# Autodesk Inventor assembly: Robot Self Driving 1
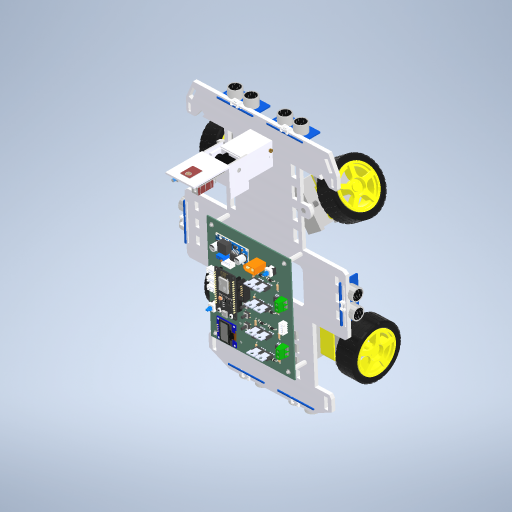
[picture p0: Inventor's stored thumbnail of the model, 512x512]
Saved by Autodesk Inventor 2023 (Build 270158000, 158)
## iProperties
Created: 2025-05-21
Part Number: Robot Self Driving 1
Document SubType Name: Assembly
Designer: ASUS
Author: ASUS
## Documents named in this file (14)
- D:\Backup C\Documents\Inventor\PMLDCAPSTONE\Robot Self Driving 1.iam
- D:\Backup C\Documents\Inventor\PMLDCAPSTONE\Robot_PMLD 1.ipt
- D:\Backup C\Documents\Inventor\PMLDCAPSTONE\Casis Kiri Roda.ipt
- D:\Backup C\Documents\Inventor\PMLDCAPSTONE\Mounting Belakang.ipt
- D:\Backup C\Documents\Inventor\PMLDCAPSTONE\RODA\Roda.iam
- D:\Backup C\Documents\Inventor\PMLDCAPSTONE\Chasis Depan Roda Kiri.ipt
- D:\Backup C\Documents\Inventor\PMLDCAPSTONE\Mounting Depan.ipt
- D:\Backup C\Documents\Inventor\PMLDCAPSTONE\Gearbox\3-6V DC Gearbox Electromotor_MIR.iam
- D:\Backup C\Documents\Inventor\PMLDCAPSTONE\standoff-male-male-m3-1.snapshot.2\3d models\Standoff M3 M-M H 20mm.ipt
- D:\Backup C\Documents\Inventor\PMLDCAPSTONE\Mur Kamera.ipt
- D:\Backup C\Documents\Inventor\PMLDCAPSTONE\Komponen PCB 1.ipt
- D:\Backup C\Documents\Inventor\PMLDCAPSTONE\Servo EMAX ES08MDII.ipt
- D:\Backup C\Documents\Inventor\PMLDCAPSTONE\Sensor Jarak\Grove_Ultrasonic_Sensor_V2.0.iam
- D:\Backup C\Documents\Inventor\PMLDCAPSTONE\fixasi\Assembly1 kamera.iam
## Components (33 placed, 13 different names)
1. Servo EMAX ES08MDII:3 — Mate:72
2. Robot_PMLD 1:2 — Mate:41, Mate:42, Mate:43, Mate:44, Mate:45, Mate:46, Mate:48, Mate:49, Mate:51, Mate:52, Mate:53, Mate:54, Mate:58, Mate:59, Mate:64, Mate:72
3. Standoff M3 M-M H 20mm:5 — Mate:41
4. Standoff M3 M-M H 20mm:6 — Mate:42, Mate:47
5. Standoff M3 M-M H 20mm:7 — Mate:43
6. Standoff M3 M-M H 20mm:8 — Mate:44
7. Mounting Depan:3 — Mate:45, Mate:73
8. Mounting Depan:4 — Mate:46, Mate:60
9. Komponen PCB 1:3 — Mate:47
10. Casis Kiri Roda:3 — Mate:48, Mate:55, Mate:69
11. Casis Kiri Roda:4 — Mate:49, Mate:50, Mate:68
12. Roda:5 [sub-assembly] — Mate:57
13. Roda:6 [sub-assembly] — Mate:56
14. Mounting Belakang:5 — Mate:50, Mate:57
15. Mounting Belakang:6 — Mate:55, Mate:56
16. Ultrasonic Ranger V2_0:7 [sub-assembly] — Mate:52
17. Ultrasonic Ranger V2_0:8 [sub-assembly] — Mate:54
18. Ultrasonic Ranger V2_0:9 [sub-assembly] — Mate:53
19. Ultrasonic Ranger V2_0:10 [sub-assembly] — Mate:51
20. Ultrasonic Ranger V2_0:11 [sub-assembly] — Mate:59
21. Ultrasonic Ranger V2_0:12 [sub-assembly] — Mate:58
22. Chasis Depan Roda Kiri:5 — Mate:60, Mate:63, Mate:76
23. 3-6V DC Gearbox Electromotor_MIR:5 [sub-assembly] — Mate:68
24. Mounting Belakang:7 — Mate:74, Mate:75
25. Mounting Belakang:8 — Mate:63, Mate:66
26. Mur Kamera:4 — Mate:64, Mate:67
27. Roda:8 [sub-assembly] — Mate:66
28. Assembly1 kamera:1 [sub-assembly] — Mate:67
29. 3-6V DC Gearbox Electromotor_MIR:8 [sub-assembly] — Mate:69
30. 3-6V DC Gearbox Electromotor_MIR:9 [sub-assembly] — Mate:76
31. Chasis Depan Roda Kiri:6 — Mate:73, Mate:74, Mate:77
32. Roda:9 [sub-assembly] — Mate:75
33. 3-6V DC Gearbox Electromotor_MIR:10 [sub-assembly] — Mate:77
## Relationships (32: Mate 32)
- Mate:41: Robot_PMLD 1:2 ↔ Standoff M3 M-M H 20mm:5
- Mate:42: Robot_PMLD 1:2 ↔ Standoff M3 M-M H 20mm:6
- Mate:43: Robot_PMLD 1:2 ↔ Standoff M3 M-M H 20mm:7
- Mate:44: Robot_PMLD 1:2 ↔ Standoff M3 M-M H 20mm:8
- Mate:45: Robot_PMLD 1:2 ↔ Mounting Depan:3
- Mate:46: Robot_PMLD 1:2 ↔ Mounting Depan:4
- Mate:47: Standoff M3 M-M H 20mm:6 ↔ Komponen PCB 1:3
- Mate:48: Robot_PMLD 1:2 ↔ Casis Kiri Roda:3
- Mate:49: Robot_PMLD 1:2 ↔ Casis Kiri Roda:4
- Mate:50: Casis Kiri Roda:4 ↔ Mounting Belakang:5
- Mate:51: Robot_PMLD 1:2 ↔ Ultrasonic Ranger V2_0:10
- Mate:52: Robot_PMLD 1:2 ↔ Ultrasonic Ranger V2_0:7
- Mate:53: Robot_PMLD 1:2 ↔ Ultrasonic Ranger V2_0:9
- Mate:54: Robot_PMLD 1:2 ↔ Ultrasonic Ranger V2_0:8
- Mate:55: Casis Kiri Roda:3 ↔ Mounting Belakang:6
- Mate:56: Roda:6 ↔ Mounting Belakang:6
- Mate:57: Roda:5 ↔ Mounting Belakang:5
- Mate:58: Robot_PMLD 1:2 ↔ Ultrasonic Ranger V2_0:12
- Mate:59: Robot_PMLD 1:2 ↔ Ultrasonic Ranger V2_0:11
- Mate:60: Mounting Depan:4 ↔ Chasis Depan Roda Kiri:5
- Mate:63: Chasis Depan Roda Kiri:5 ↔ Mounting Belakang:8
- Mate:64: Robot_PMLD 1:2 ↔ Mur Kamera:4
- Mate:66: Mounting Belakang:8 ↔ Roda:8
- Mate:67: Mur Kamera:4 ↔ Assembly1 kamera:1
- Mate:68: Casis Kiri Roda:4 ↔ 3-6V DC Gearbox Electromotor_MIR:5
- Mate:69: Casis Kiri Roda:3 ↔ 3-6V DC Gearbox Electromotor_MIR:8
- Mate:72: Servo EMAX ES08MDII:3 ↔ Robot_PMLD 1:2
- Mate:73: Mounting Depan:3 ↔ Chasis Depan Roda Kiri:6
- Mate:74: Mounting Belakang:7 ↔ Chasis Depan Roda Kiri:6
- Mate:75: Mounting Belakang:7 ↔ Roda:9
- Mate:76: Chasis Depan Roda Kiri:5 ↔ 3-6V DC Gearbox Electromotor_MIR:9
- Mate:77: Chasis Depan Roda Kiri:6 ↔ 3-6V DC Gearbox Electromotor_MIR:10
